# Autodesk Inventor assembly: FinalRobot
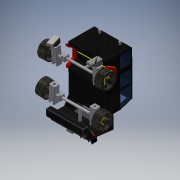
[picture p0: Inventor's stored thumbnail of the model, 180x180]
Saved by Autodesk Inventor 2017 (Build 210142000, 142)
## iProperties
Part Number: FinalRobot
Material: Genérico
Document SubType Name: Assembly
Designer: Ghost
Author: Ghost
## Documents named in this file (9)
- C:\Users\Ghost\Desktop\UVG Semestre 8\Dibujo Mecanico\ProyectoTransformer\FinalRobot.iam
- C:\Users\Ghost\Desktop\UVG Semestre 8\Dibujo Mecanico\ProyectoTransformer\ProyectoTransformer\Ante pierna.ipt
- C:\Users\Ghost\Desktop\UVG Semestre 8\Dibujo Mecanico\ProyectoTransformer\ProyectoTransformer\Union pie.ipt
- C:\Users\Ghost\Desktop\UVG Semestre 8\Dibujo Mecanico\ProyectoTransformer\ProyectoTransformer\Hombro.ipt
- C:\Users\Ghost\Desktop\UVG Semestre 8\Dibujo Mecanico\ProyectoTransformer\ProyectoTransformer\llanta.ipt
- C:\Users\Ghost\Desktop\UVG Semestre 8\Dibujo Mecanico\ProyectoTransformer\ProyectoTransformer\Bumper.ipt
- C:\Users\Ghost\Desktop\UVG Semestre 8\Dibujo Mecanico\ProyectoTransformer\ProyectoTransformer\CabezaCarro.ipt
- C:\Users\Ghost\Desktop\UVG Semestre 8\Dibujo Mecanico\ProyectoTransformer\ProyectoTransformer\PuertaMarco.iam
- C:\Users\Ghost\Desktop\UVG Semestre 8\Dibujo Mecanico\ProyectoTransformer\ProyectoTransformer\Pie.ipt
## Components (23 placed, 8 different names)
1. Ante pierna:1 — Coincidencia:1, Coincidencia:2, Coincidencia:3, Coincidencia:6, Coincidencia:7
2. Union pie:1 — Coincidencia:1, Coincidencia:2, Coincidencia:3, Coincidencia:4, Coincidencia:5
3. Hombro:1 — Coincidencia:4, Coincidencia:5, Coincidencia:8, Coincidencia:9
4. llanta:1 — Coincidencia:6, Coincidencia:7
5. Bumper:1 — Coincidencia:8, Coincidencia:9, Coincidencia:10, Coincidencia:11, Coincidencia:20, Coincidencia:21, Insertar:1, Insertar:2
6. Union pie:2 — Coincidencia:12, Coincidencia:13, Coincidencia:14, Coincidencia:15, Coincidencia:16, Coincidencia:17
7. Ante pierna:2 — Coincidencia:14, Coincidencia:15, Coincidencia:16, Coincidencia:17, Coincidencia:18, Coincidencia:19
8. Hombro:2 — Coincidencia:10, Coincidencia:11, Coincidencia:12, Coincidencia:13
9. llanta:2 — Coincidencia:18, Coincidencia:19
10. CabezaCarro:1 — Coincidencia:20, Coincidencia:21
11. PuertaMarco:1 [sub-assembly] — Insertar:1, Insertar:2, Insertar:3, Insertar:6
12. Ante pierna:3 — Coincidencia:22, Coincidencia:23, Insertar:7, Insertar:9
13. Union pie:3 — Insertar:4, Coincidencia:22, Coincidencia:23
14. llanta:3 — Insertar:7
15. Hombro:3 — Insertar:3, Insertar:4
16. Hombro:4 — Insertar:5, Insertar:6
17. Ante pierna:4 — Coincidencia:24, Coincidencia:25, Insertar:8, Insertar:10
18. Union pie:4 — Insertar:5, Coincidencia:24, Coincidencia:25
19. llanta:4 — Insertar:8
20. Pie:1 — Coincidencia:26, Coincidencia:27
21. Pie:2 — Coincidencia:28, Coincidencia:29
22. Union pie:5 — Insertar:9, Coincidencia:26, Coincidencia:27
23. Union pie:6 — Insertar:10, Coincidencia:28, Coincidencia:29
## Relationships (39: Mate 29, Insert 10)
- Coincidencia:1 [Mate]: Ante pierna:1 ↔ Union pie:1
- Coincidencia:2 [Mate]: Ante pierna:1 ↔ Union pie:1
- Coincidencia:3 [Mate]: Ante pierna:1 ↔ Union pie:1
- Coincidencia:4 [Mate]: Union pie:1 ↔ Hombro:1
- Coincidencia:5 [Mate]: Union pie:1 ↔ Hombro:1
- Coincidencia:6 [Mate]: Ante pierna:1 ↔ llanta:1
- Coincidencia:7 [Mate]: Ante pierna:1 ↔ llanta:1
- Coincidencia:8 [Mate]: Hombro:1 ↔ Bumper:1
- Coincidencia:9 [Mate]: Hombro:1 ↔ Bumper:1
- Coincidencia:10 [Mate]: Bumper:1 ↔ Hombro:2
- Coincidencia:11 [Mate]: Bumper:1 ↔ Hombro:2
- Coincidencia:12 [Mate]: Union pie:2 ↔ Hombro:2
- Coincidencia:13 [Mate]: Union pie:2 ↔ Hombro:2
- Coincidencia:14 [Mate]: Union pie:2 ↔ Ante pierna:2
- Coincidencia:15 [Mate]: Union pie:2 ↔ Ante pierna:2
- Coincidencia:16 [Mate]: Union pie:2 ↔ Ante pierna:2
- Coincidencia:17 [Mate]: Union pie:2 ↔ Ante pierna:2
- Coincidencia:18 [Mate]: Ante pierna:2 ↔ llanta:2
- Coincidencia:19 [Mate]: Ante pierna:2 ↔ llanta:2
- Coincidencia:20 [Mate]: Bumper:1 ↔ CabezaCarro:1
- Coincidencia:21 [Mate]: Bumper:1 ↔ CabezaCarro:1
- Insertar:1: Bumper:1 ↔ PuertaMarco:1
- Insertar:2: Bumper:1 ↔ PuertaMarco:1
- Insertar:3: PuertaMarco:1 ↔ Hombro:3
- Insertar:4: Union pie:3 ↔ Hombro:3
- Coincidencia:22 [Mate]: Ante pierna:3 ↔ Union pie:3
- Coincidencia:23 [Mate]: Ante pierna:3 ↔ Union pie:3
- Insertar:5: Hombro:4 ↔ Union pie:4
- Insertar:6: PuertaMarco:1 ↔ Hombro:4
- Coincidencia:24 [Mate]: Ante pierna:4 ↔ Union pie:4
- Coincidencia:25 [Mate]: Ante pierna:4 ↔ Union pie:4
- Insertar:7: Ante pierna:3 ↔ llanta:3
- Insertar:8: Ante pierna:4 ↔ llanta:4
- Insertar:9: Ante pierna:3 ↔ Union pie:5
- Coincidencia:26 [Mate]: Pie:1 ↔ Union pie:5
- Coincidencia:27 [Mate]: Pie:1 ↔ Union pie:5
- Insertar:10: Ante pierna:4 ↔ Union pie:6
- Coincidencia:28 [Mate]: Pie:2 ↔ Union pie:6
- Coincidencia:29 [Mate]: Pie:2 ↔ Union pie:6
